# Autodesk Inventor assembly: X_GANTRY
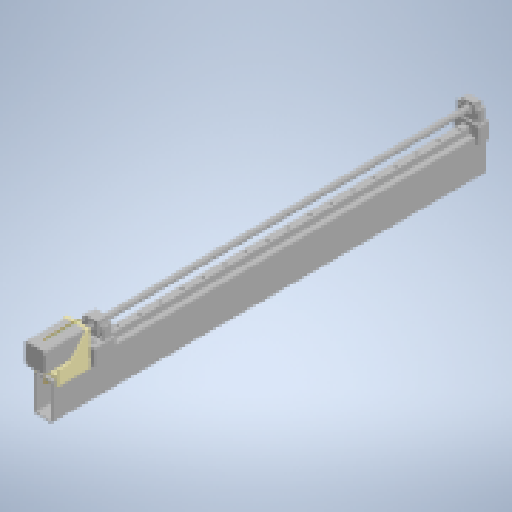
[picture p0: Inventor's stored thumbnail of the model, 512x512]
Saved by Autodesk Inventor 2023 (Build 270158000, 158)
## iProperties
Created: 2022-05-04
Part Number: X_GANTRY
Document SubType Name: Assembly
Designer: plebbb
Author: plebbb
## Documents named in this file (12)
- C:\Users\think\OneDrive\Desktop\CNC_Project\X_GANTRY.iam
- C:\Users\think\OneDrive\Desktop\CNC_Project\2x3_Tube.ipt
- C:\Users\think\OneDrive\Desktop\CNC_Project\HGW20CC_Rail_800mm.ipt
- C:\Users\think\OneDrive\Desktop\CNC_Project\SFU1605_800mm.ipt
- C:\Users\think\OneDrive\Desktop\CNC_Project\BF12.ipt
- C:\Users\think\OneDrive\Desktop\CNC_Project\BK12.ipt
- C:\Users\think\OneDrive\Desktop\CNC_Project\BK12_Spacer.ipt
- C:\Users\think\OneDrive\Desktop\CNC_Project\BF12_Spacer.ipt
- C:\Users\think\OneDrive\Desktop\CNC_Project\Nema23.ipt
- C:\Users\think\OneDrive\Desktop\CNC_Project\Nema23_Mount.ipt
- C:\Users\think\OneDrive\Desktop\CNC_Project\Sensor_Adapter_v2.ipt
- C:\Users\think\OneDrive\Desktop\CNC_Project\LJ12.ipt
## Components (11 placed, 11 different names)
1. 2x3_Tube:1 — Mate:16, Mate:17, Flush:3, Flush:4, Mate:18, Mate:23, Mate:30, Flush:5, Mate:33, Mate:34
2. HGW20CC_Rail_800mm:1 — Flush:4, Mate:18, Mate:31
3. SFU1605_800mm:1 — Mate:24, Mate:35
4. BF12:1 — Mate:29, Mate:32
5. BK12:1 — Flush:6, Mate:38, Mate:39
6. BK12_Spacer:1 — Mate:34
7. BF12_Spacer:1 — Mate:29, Mate:30, Mate:31, Flush:5, Mate:32
8. Nema23:1 — Mate:35, Mate:36, Mate:37
9. Nema23_Mount:1 — Mate:23, Mate:24, Mate:33, Mate:36, Mate:37
10. Sensor_Adapter_v2:1 — Flush:6, Mate:38, Mate:39, Mate:40
11. LJ12:1 — Mate:40
## Relationships (28: Mate 23, Flush 5)
- [Mate]: SFU1605_800mm:1 ↔ BK12:1
- [Flush]: SFU1605_800mm:1 ↔ BK12:1
- [Mate]: SFU1605_800mm:1 ↔ BF12:1
- [Mate]: SFU1605_800mm:1 ↔ BF12:1
- [Mate]: BK12:1 ↔ BK12_Spacer:1
- [Mate]: BK12:1 ↔ BK12_Spacer:1
- [Mate]: BK12:1 ↔ BK12_Spacer:1
- Mate:16: 2x3_Tube:1
- Mate:17: 2x3_Tube:1
- Flush:3: 2x3_Tube:1
- Flush:4 (15.4 mm): 2x3_Tube:1 ↔ HGW20CC_Rail_800mm:1
- Mate:18: 2x3_Tube:1 ↔ HGW20CC_Rail_800mm:1
- Mate:23: 2x3_Tube:1 ↔ Nema23_Mount:1
- Mate:24: SFU1605_800mm:1 ↔ Nema23_Mount:1
- Mate:29: BF12:1 ↔ BF12_Spacer:1
- Mate:30: 2x3_Tube:1 ↔ BF12_Spacer:1
- Mate:31: HGW20CC_Rail_800mm:1 ↔ BF12_Spacer:1
- Flush:5: 2x3_Tube:1 ↔ BF12_Spacer:1
- Mate:32: BF12:1 ↔ BF12_Spacer:1
- Mate:33 (0.25 mm): 2x3_Tube:1 ↔ Nema23_Mount:1
- Mate:34 (0.25 mm): 2x3_Tube:1 ↔ BK12_Spacer:1
- Mate:35: SFU1605_800mm:1 ↔ Nema23:1
- Mate:36: Nema23:1 ↔ Nema23_Mount:1
- Mate:37: Nema23:1 ↔ Nema23_Mount:1
- Flush:6: BK12:1 ↔ Sensor_Adapter_v2:1
- Mate:38: BK12:1 ↔ Sensor_Adapter_v2:1
- Mate:39: BK12:1 ↔ Sensor_Adapter_v2:1
- Mate:40: Sensor_Adapter_v2:1 ↔ LJ12:1
